# Autodesk Inventor assembly: Leg_joint_roll_pitch
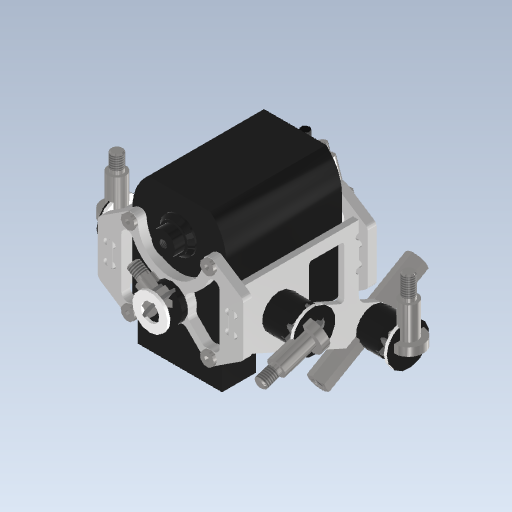
[picture p0: Inventor's stored thumbnail of the model, 512x512]
Saved by Autodesk Inventor 2020.4 (Build 244396000, 396)
## iProperties
Part Number: Leg_joint_roll_pitch
Document SubType Name: Assembly
Designer: Masato Kubotera
Mass: 101.309 g
Surface Area: 368.925 cm^2
Volume: 74.117 cm^3
Density: 1.36688 g/cm^3
Author: Masato Kubotera
## Documents named in this file (22)
- C:\Users\Masato\Documents\Inventor\CIT Brains_Inventor\OpenPlatform_ver3_0\LowerBody\Leg_joit\Leg_joint_roll_pitch.iam
- C:\Users\Masato\Documents\Inventor\CIT Brains_Inventor\OpenPlatform_ver3_0\LowerBody\Leg_joit\Leg_joint_pitch_frame.ipt
- C:\Users\Masato\Documents\Inventor\CIT Brains_Inventor\OpenPlatform_ver3_0\LowerBody\Leg_joit\Leg_joint_roll_frame.ipt
- C:\Users\Masato\Documents\Inventor\CIT Brains_Inventor\OpenPlatform_ver3_0\ReadyMade\KONDO\B3M-SC-1170-A.ipt
- C:\Users\Masato\Documents\Inventor\CIT Brains_Inventor\OpenPlatform_ver3_0\ReadyMade\Screw\M2_6-20.ipt
- C:\Users\Masato\Documents\Inventor\CIT Brains_Inventor\OpenPlatform_ver3_0\ReadyMade\Screw\M2_6-15.ipt
- C:\Users\Masato\Documents\Inventor\CIT Brains_Inventor\OpenPlatform_ver3_0\ReadyMade\Bush\80F-0603.ipt
- C:\Users\Masato\Documents\Inventor\CIT Brains_Inventor\OpenPlatform_ver3_0\ReadyMade\Washer\CC-0612-15B.ipt
- C:\Users\Masato\Documents\Inventor\CIT Brains_Inventor\OpenPlatform_ver3_0\ReadyMade\Washer\CC-0612-50B.ipt
- C:\Users\Masato\Documents\Inventor\CIT Brains_Inventor\OpenPlatform_ver3_0\ReadyMade\InsertNut\SF419.ipt
- C:\Users\Masato\Documents\Inventor\CIT Brains_Inventor\OpenPlatform_ver3_0\ReadyMade\Washer\UUW-0412-10BH.ipt
- C:\Users\Masato\Documents\Inventor\CIT Brains_Inventor\OpenPlatform_ver3_0\ReadyMade\Spacer\SLSBF6-39.5-M4-N4.ipt
- C:\Users\Masato\Documents\Inventor\CIT Brains_Inventor\OpenPlatform_ver3_0\ReadyMade\Screw\DBTS4-11-6.ipt
- C:\Users\Masato\Documents\Inventor\CIT Brains_Inventor\OpenPlatform_ver3_0\ReadyMade\Screw\DBS4-5-5.ipt
- C:\Users\Masato\Documents\Inventor\CIT Brains_Inventor\OpenPlatform_ver3_0\ReadyMade\Screw\DBTS4-10-4.ipt
- C:\Users\Masato\Documents\Inventor\CIT Brains_Inventor\OpenPlatform_ver3_0\ReadyMade\InsertNut\S4-05-3W.ipt
- C:\Users\Masato\Documents\Inventor\CIT Brains_Inventor\OpenPlatform_ver3_0\ReadyMade\KONDO\ClampHorn.ipt
- C:\Users\Masato\Documents\Inventor\CIT Brains_Inventor\OpenPlatform_ver3_0\ReadyMade\Screw\620103008.ipt
- C:\Users\Masato\Documents\Inventor\CIT Brains_Inventor\OpenPlatform_ver3_0\ReadyMade\Screw\DBTS4-11-8.ipt
- C:\Users\Masato\Documents\Inventor\CIT Brains_Inventor\OpenPlatform_ver3_0\ReadyMade\Washer\UUW-0614-05BH.ipt
- C:\Users\Masato\Documents\Inventor\CIT Brains_Inventor\OpenPlatform_ver3_0\ReadyMade\Washer\TT-0612-10.ipt
- C:\Users\Masato\Documents\Inventor\CIT Brains_Inventor\OpenPlatform_ver3_0\ReadyMade\Washer\TT-0814-10.ipt
## Components (56 placed, 21 different names)
1. B3M-SC-1170-A:1 — 挿入:1, 挿入:2, 挿入:3, 挿入:4, 挿入:11, 挿入:12, 挿入:13, 挿入:14, メイト:1, メイト:2, フラッシュ:1, 挿入:49, 角度:3
2. Leg_joint_roll_frame:1 — 挿入:1, 挿入:2, 挿入:3, 挿入:4, 挿入:5, 挿入:6, 挿入:7, 挿入:8, 挿入:9, 挿入:10, 角度:1, フラッシュ:2, メイト:3, メイト:4, メイト:5
3. Leg_joint_roll_frame:2 — 挿入:11, 挿入:12, 挿入:13, 挿入:14, 挿入:15, 挿入:16, 挿入:17, 挿入:18, 角度:2, 角度:4
4. Leg_joint_pitch_frame:1 — フラッシュ:3, 挿入:19, フラッシュ:4, メイト:5, 挿入:20, 挿入:21, 挿入:22
5. Leg_joint_pitch_frame:2 — フラッシュ:2, フラッシュ:3, フラッシュ:4, メイト:3, メイト:4, 挿入:23, 挿入:24, 挿入:25, 挿入:26
6. M2_6-20:1 — 挿入:7
7. M2_6-20:2 — 挿入:8
8. M2_6-20:3 — 挿入:5
9. M2_6-20:4 — 挿入:6
10. M2_6-15:2 — 挿入:16
11. M2_6-15:3 — 挿入:15
12. 80F-0603:1 — 挿入:43
13. 80F-0603:2 — 挿入:44
14. 80F-0603:3 — 挿入:45
15. 80F-0603:4 — 挿入:46
16. 80F-0603:5 — 挿入:47
17. 80F-0603:6 — 挿入:48
18. UUW-0412-10BH:1 — 挿入:9, 挿入:27
19. UUW-0412-10BH:2 — 挿入:17, 挿入:28, 挿入:33
20. UUW-0412-10BH:3 — 挿入:19, 挿入:29, 挿入:226
21. UUW-0412-10BH:4 — 挿入:22, 挿入:30, 挿入:35
22. UUW-0412-10BH:5 — 挿入:23, 挿入:31, 挿入:227
23. UUW-0412-10BH:6 — 挿入:26, 挿入:32, 挿入:37
24. UUW-0412-10BH:7 — 挿入:27, 挿入:38, 挿入:43
25. CC-0612-15B:1 — 挿入:29, 挿入:39
26. CC-0612-15B:2 — 挿入:30, 挿入:40
27. CC-0612-15B:3 — 挿入:31, 挿入:41
28. CC-0612-15B:4 — 挿入:32, 挿入:42
29. CC-0612-50B:1 — 挿入:39, 挿入:45
30. CC-0612-50B:2 — 挿入:40, 挿入:46
31. CC-0612-50B:3 — 挿入:41, 挿入:47
32. CC-0612-50B:4 — 挿入:42, 挿入:48
33. CC-0612-50B:5 — 挿入:28, 挿入:44
34. SF419:1 — 挿入:25
35. SF419:2 — 挿入:20
36. S4-05-3W:1 — 挿入:10, 角度:1
37. S4-05-3W:2 — 挿入:18, 角度:2
38. SLSBF6-39.5-M4-N4:1 — 挿入:21, 挿入:24, 角度:4
39. DBS4-5-5:1 — 挿入:38, 挿入:232
40. DBTS4-11-6:3 — 挿入:37, 挿入:229
41. DBTS4-11-6:4 — 挿入:35, 挿入:230
42. DBTS4-10-4:1 — 挿入:33, 挿入:233
43. ClampHorn:1 — 挿入:49, 挿入:50, 角度:3
44. 620103008:1 — 挿入:50
45. DBTS4-11-8:1 — 挿入:226, 挿入:231
46. DBTS4-11-8:2 — 挿入:227, 挿入:228
47. UUW-0614-05BH:1 — 挿入:228, 挿入:234
48. UUW-0614-05BH:2 — 挿入:229, 挿入:235
49. UUW-0614-05BH:3 — 挿入:230, 挿入:236
50. UUW-0614-05BH:4 — 挿入:231, 挿入:237
51. TT-0612-10:1 — 挿入:233
52. TT-0612-10:2 — 挿入:232
53. TT-0814-10:1 — 挿入:234
54. TT-0814-10:2 — 挿入:235
55. TT-0814-10:3 — 挿入:237
56. TT-0814-10:4 — 挿入:236
## Relationships (73: Insert 60, Mate 5, Flush 4, Angle 4)
- フラッシュ:1 [Flush]: B3M-SC-1170-A:1
- メイト:1 [Mate]: B3M-SC-1170-A:1
- メイト:2 [Mate]: B3M-SC-1170-A:1
- 挿入:1 [Insert]: B3M-SC-1170-A:1 ↔ Leg_joint_roll_frame:1
- 挿入:2 [Insert]: B3M-SC-1170-A:1 ↔ Leg_joint_roll_frame:1
- 挿入:3 [Insert]: B3M-SC-1170-A:1 ↔ Leg_joint_roll_frame:1
- 挿入:4 [Insert]: B3M-SC-1170-A:1 ↔ Leg_joint_roll_frame:1
- 挿入:5 [Insert]: Leg_joint_roll_frame:1 ↔ M2_6-20:3
- 挿入:6 [Insert]: Leg_joint_roll_frame:1 ↔ M2_6-20:4
- 挿入:7 [Insert]: Leg_joint_roll_frame:1 ↔ M2_6-20:1
- 挿入:8 [Insert]: Leg_joint_roll_frame:1 ↔ M2_6-20:2
- 挿入:9 [Insert]: Leg_joint_roll_frame:1 ↔ UUW-0412-10BH:1
- 挿入:10 [Insert]: Leg_joint_roll_frame:1 ↔ S4-05-3W:1
- 角度:1 [Angle] (0 deg): Leg_joint_roll_frame:1 ↔ S4-05-3W:1
- 挿入:11 [Insert]: B3M-SC-1170-A:1 ↔ Leg_joint_roll_frame:2
- 挿入:12 [Insert]: B3M-SC-1170-A:1 ↔ Leg_joint_roll_frame:2
- 挿入:13 [Insert]: B3M-SC-1170-A:1 ↔ Leg_joint_roll_frame:2
- 挿入:14 [Insert]: B3M-SC-1170-A:1 ↔ Leg_joint_roll_frame:2
- 挿入:15 [Insert]: Leg_joint_roll_frame:2 ↔ M2_6-15:3
- 挿入:16 [Insert]: Leg_joint_roll_frame:2 ↔ M2_6-15:2
- 挿入:17 [Insert]: Leg_joint_roll_frame:2 ↔ UUW-0412-10BH:2
- 挿入:18 [Insert]: Leg_joint_roll_frame:2 ↔ S4-05-3W:2
- 角度:2 [Angle] (0 deg): Leg_joint_roll_frame:2 ↔ S4-05-3W:2
- 挿入:19 [Insert]: Leg_joint_pitch_frame:1 ↔ UUW-0412-10BH:3
- 挿入:20 [Insert]: Leg_joint_pitch_frame:1 ↔ SF419:2
- 挿入:21 [Insert]: Leg_joint_pitch_frame:1 ↔ SLSBF6-39.5-M4-N4:1
- 挿入:22 [Insert]: Leg_joint_pitch_frame:1 ↔ UUW-0412-10BH:4
- 挿入:23 [Insert]: Leg_joint_pitch_frame:2 ↔ UUW-0412-10BH:5
- 挿入:24 [Insert]: Leg_joint_pitch_frame:2 ↔ SLSBF6-39.5-M4-N4:1
- 挿入:25 [Insert]: Leg_joint_pitch_frame:2 ↔ SF419:1
- 挿入:26 [Insert]: Leg_joint_pitch_frame:2 ↔ UUW-0412-10BH:6
- 挿入:27 [Insert]: UUW-0412-10BH:1 ↔ UUW-0412-10BH:7
- 挿入:28 [Insert]: UUW-0412-10BH:2 ↔ CC-0612-50B:5
- 挿入:29 [Insert]: UUW-0412-10BH:3 ↔ CC-0612-15B:1
- 挿入:30 [Insert]: UUW-0412-10BH:4 ↔ CC-0612-15B:2
- 挿入:31 [Insert]: UUW-0412-10BH:5 ↔ CC-0612-15B:3
- 挿入:32 [Insert]: UUW-0412-10BH:6 ↔ CC-0612-15B:4
- 挿入:33 [Insert]: UUW-0412-10BH:2 ↔ DBTS4-10-4:1
- 挿入:35 [Insert]: UUW-0412-10BH:4 ↔ DBTS4-11-6:4
- 挿入:37 [Insert]: UUW-0412-10BH:6 ↔ DBTS4-11-6:3
- 挿入:38 [Insert]: UUW-0412-10BH:7 ↔ DBS4-5-5:1
- 挿入:39 [Insert]: CC-0612-15B:1 ↔ CC-0612-50B:1
- 挿入:40 [Insert]: CC-0612-15B:2 ↔ CC-0612-50B:2
- 挿入:41 [Insert]: CC-0612-15B:3 ↔ CC-0612-50B:3
- 挿入:42 [Insert]: CC-0612-15B:4 ↔ CC-0612-50B:4
- 挿入:43 [Insert]: 80F-0603:1 ↔ UUW-0412-10BH:7
- 挿入:44 [Insert]: 80F-0603:2 ↔ CC-0612-50B:5
- 挿入:45 [Insert]: 80F-0603:3 ↔ CC-0612-50B:1
- 挿入:46 [Insert]: 80F-0603:4 ↔ CC-0612-50B:2
- 挿入:47 [Insert]: 80F-0603:5 ↔ CC-0612-50B:3
- 挿入:48 [Insert]: 80F-0603:6 ↔ CC-0612-50B:4
- フラッシュ:2 [Flush]: Leg_joint_roll_frame:1 ↔ Leg_joint_pitch_frame:2
- フラッシュ:3 [Flush]: Leg_joint_pitch_frame:1 ↔ Leg_joint_pitch_frame:2
- フラッシュ:4 [Flush]: Leg_joint_pitch_frame:1 ↔ Leg_joint_pitch_frame:2
- メイト:3 [Mate] (0.025 mm): Leg_joint_roll_frame:1 ↔ Leg_joint_pitch_frame:2
- メイト:4 [Mate] (0.025 mm): Leg_joint_roll_frame:1 ↔ Leg_joint_pitch_frame:2
- メイト:5 [Mate] (0.025 mm): Leg_joint_roll_frame:1 ↔ Leg_joint_pitch_frame:1
- 挿入:49 [Insert]: B3M-SC-1170-A:1 ↔ ClampHorn:1
- 挿入:50 [Insert]: ClampHorn:1 ↔ 620103008:1
- 角度:3 [Angle] (0 deg): B3M-SC-1170-A:1 ↔ ClampHorn:1
- 角度:4 [Angle] (0 deg): Leg_joint_roll_frame:2 ↔ SLSBF6-39.5-M4-N4:1
- 挿入:226 [Insert]: UUW-0412-10BH:3 ↔ DBTS4-11-8:1
- 挿入:227 [Insert]: UUW-0412-10BH:5 ↔ DBTS4-11-8:2
- 挿入:228 [Insert]: DBTS4-11-8:2 ↔ UUW-0614-05BH:1
- 挿入:229 [Insert]: DBTS4-11-6:3 ↔ UUW-0614-05BH:2
- 挿入:230 [Insert]: DBTS4-11-6:4 ↔ UUW-0614-05BH:3
- 挿入:231 [Insert]: DBTS4-11-8:1 ↔ UUW-0614-05BH:4
- 挿入:232 [Insert]: DBS4-5-5:1 ↔ TT-0612-10:2
- 挿入:233 [Insert]: DBTS4-10-4:1 ↔ TT-0612-10:1
- 挿入:234 [Insert]: UUW-0614-05BH:1 ↔ TT-0814-10:1
- 挿入:235 [Insert]: UUW-0614-05BH:2 ↔ TT-0814-10:2
- 挿入:236 [Insert]: UUW-0614-05BH:3 ↔ TT-0814-10:4
- 挿入:237 [Insert]: UUW-0614-05BH:4 ↔ TT-0814-10:3
